# Autodesk Inventor assembly: CNC
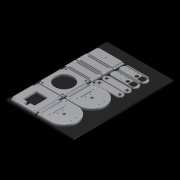
[picture p0: Inventor's stored thumbnail of the model, 180x180]
Saved by Autodesk Inventor 2011 (Build 150239000, 239)
## iProperties
Created: 2012-11-29
Part Number: CNC
Document SubType Name: Assembly
Designer: arihon
Author: arihon
## Documents named in this file (10)
- C:\Users\JohnHenry\Dropbox\Inventor\walkPivot\CNC.iam
- C:\Users\JohnHenry\Dropbox\Inventor\walkPivot\CNC.ipt
- C:\Users\JohnHenry\Dropbox\Inventor\walkPivot\JointA1.ipt
- C:\Users\JohnHenry\Dropbox\Inventor\walkPivot\JointA2.ipt
- C:\Users\JohnHenry\Dropbox\Inventor\walkPivot\JointA3.ipt
- C:\Users\JohnHenry\Dropbox\Inventor\walkPivot\JointB1.ipt
- C:\Users\JohnHenry\Dropbox\Inventor\walkPivot\JointB2.ipt
- C:\Users\JohnHenry\Dropbox\Inventor\walkPivot\JointC2_.ipt
- C:\Users\JohnHenry\Dropbox\Inventor\walkPivot\JointC4.ipt
- C:\Users\JohnHenry\Dropbox\Inventor\walkPivot\JointD0.ipt
## Components (12 placed, 9 different names)
1. CNC:1 — メイト:1, メイト:2, メイト:3, メイト:4, メイト:5, メイト:6, メイト:7, メイト:9, メイト:10, メイト:11, フラッシュ:6, フラッシュ:7, フラッシュ:8, メイト:22
2. JointA1:1 — メイト:1, フラッシュ:1, フラッシュ:6, フラッシュ:7, メイト:13, メイト:17
3. JointA2:1 — メイト:2, フラッシュ:1, フラッシュ:2, メイト:13, メイト:14
4. JointA3:1 — メイト:3, フラッシュ:2, フラッシュ:3, メイト:14, メイト:15, 正接:1, 正接:5
5. JointA3:2 — メイト:4, フラッシュ:3, フラッシュ:4, メイト:15, メイト:16, 正接:3
6. JointB1:1 — メイト:6, フラッシュ:5, メイト:12, フラッシュ:8
7. JointB1:2 — メイト:5, フラッシュ:5, メイト:12, メイト:17, メイト:18
8. JointB2:1 — メイト:7, フラッシュ:4, メイト:16, 正接:4
9. JointC2_:1 — メイト:9, メイト:11, メイト:21, 正接:4
10. JointC4:1 — メイト:10, メイト:18, 正接:1, メイト:23
11. JointD0:1 — メイト:21, 正接:3, メイト:24
12. JointC4:2 — メイト:22, メイト:23, メイト:24, 正接:5
## Relationships (33: Mate 21, Flush 8, Tangent 4)
- メイト:1 [Mate]: CNC:1 ↔ JointA1:1
- メイト:2 [Mate]: CNC:1 ↔ JointA2:1
- メイト:3 [Mate]: CNC:1 ↔ JointA3:1
- メイト:4 [Mate]: CNC:1 ↔ JointA3:2
- メイト:5 [Mate]: CNC:1 ↔ JointB1:2
- メイト:6 [Mate]: CNC:1 ↔ JointB1:1
- メイト:7 [Mate]: CNC:1 ↔ JointB2:1
- メイト:9 [Mate]: CNC:1 ↔ JointC2_:1
- メイト:10 [Mate]: CNC:1 ↔ JointC4:1
- メイト:11 [Mate]: CNC:1 ↔ JointC2_:1
- フラッシュ:1 [Flush]: JointA1:1 ↔ JointA2:1
- フラッシュ:2 [Flush]: JointA2:1 ↔ JointA3:1
- フラッシュ:3 [Flush]: JointA3:1 ↔ JointA3:2
- フラッシュ:4 [Flush]: JointA3:2 ↔ JointB2:1
- フラッシュ:5 [Flush]: JointB1:1 ↔ JointB1:2
- フラッシュ:6 [Flush] (5 mm): CNC:1 ↔ JointA1:1
- フラッシュ:7 [Flush] (5 mm): CNC:1 ↔ JointA1:1
- メイト:12 [Mate] (3 mm): JointB1:1 ↔ JointB1:2
- メイト:13 [Mate] (3 mm): JointA1:1 ↔ JointA2:1
- メイト:14 [Mate] (3 mm): JointA2:1 ↔ JointA3:1
- メイト:15 [Mate] (3 mm): JointA3:1 ↔ JointA3:2
- メイト:16 [Mate] (3 mm): JointA3:2 ↔ JointB2:1
- メイト:17 [Mate] (3 mm): JointA1:1 ↔ JointB1:2
- フラッシュ:8 [Flush] (5 mm): CNC:1 ↔ JointB1:1
- メイト:18 [Mate] (3 mm): JointB1:2 ↔ JointC4:1
- メイト:21 [Mate] (3 mm): JointC2_:1 ↔ JointD0:1
- 正接:1 [Tangent] (3 mm): JointA3:1 ↔ JointC4:1
- 正接:3 [Tangent] (3 mm): JointA3:2 ↔ JointD0:1
- 正接:4 [Tangent] (3 mm): JointB2:1 ↔ JointC2_:1
- メイト:22 [Mate]: CNC:1 ↔ JointC4:2
- メイト:23 [Mate] (3 mm): JointC4:1 ↔ JointC4:2
- メイト:24 [Mate] (3 mm): JointD0:1 ↔ JointC4:2
- 正接:5 [Tangent] (3 mm): JointA3:1 ↔ JointC4:2
